# Autodesk Inventor assembly: wheel
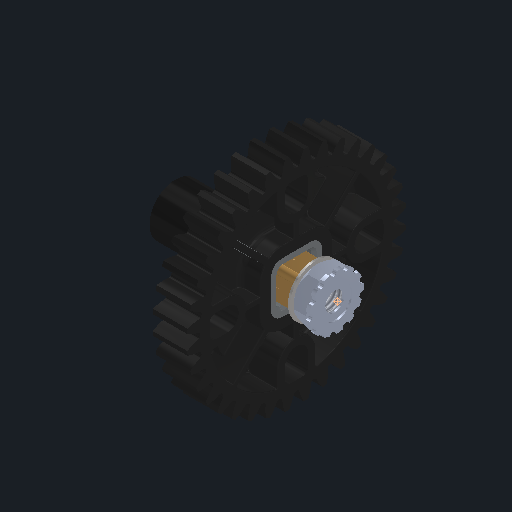
[picture p0: Inventor's stored thumbnail of the model, 512x512]
Saved by Autodesk Inventor 2025 (Build 290162000, 162)
## iProperties
Created: 2024-10-11
Part Number: wheel
Document SubType Name: Assembly
Designer: Averey Ku
Author: Averey Ku
## Documents named in this file (8)
- D:\vex_robotics_high_stakes\hardware\cad\bots\high_stakes_v2\chassis_v2\drivebay\iidler.iam
- D:\vex_robotics_high_stakes\hardware\cad\robpros_cad_lib\Modified Parts\modified_parts\Half Cut HS 36T Gear, No Insert.ipt
- D:\vex_robotics_high_stakes\hardware\cad\robpros_cad_lib\Motion\HS Shaft Adapter Circle.ipt
- D:\vex_robotics_high_stakes\hardware\cad\robpros_cad_lib\Structure\Hardware\Nut Keps.ipt
- D:\vex_robotics_high_stakes\hardware\cad\robpros_cad_lib\Motion\Spacers\Washer Steel\SWasher .375 OD x .015625.ipt
- D:\vex_robotics_high_stakes\hardware\cad\robpros_cad_lib\Motion\Spacers\Washer Steel.ipt
- D:\vex_robotics_high_stakes\hardware\cad\VEX-CAD-Inventor\Motion\Spacers\Spacer Nylon .375 OD\NSpacer .375 OD x .500.ipt
- D:\vex_robotics_high_stakes\hardware\cad\VEX-CAD-Inventor\Motion\Spacers\Spacer Nylon .375 OD.ipt
## Components (5 placed, 5 different names)
1. Half Cut HS 36T Gear, No Insert:1 — Insert:3, Insert:6
2. HS Shaft Adapter Circle:1 — Insert:3, Insert:8
3. Nut Keps:1 — Mate:1, Insert:9
4. SWasher .375 OD x .015625:2 — Insert:6, Insert:9
5. NSpacer .375 OD x .500:1 — Insert:8
## Relationships (6: Insert 4, Angle 1, Mate 1)
- Insert:3 (-3.175 mm): Half Cut HS 36T Gear, No Insert:1 ↔ HS Shaft Adapter Circle:1
- [Angle] (0 deg): Half Cut HS 36T Gear, No Insert:1 ↔ HS Shaft Adapter Circle:1
- Insert:6 (3.175 mm): Half Cut HS 36T Gear, No Insert:1 ↔ SWasher .375 OD x .015625:2
- Mate:1: Nut Keps:1
- Insert:8: HS Shaft Adapter Circle:1 ↔ NSpacer .375 OD x .500:1
- Insert:9: Nut Keps:1 ↔ SWasher .375 OD x .015625:2
